# Autodesk Inventor assembly: launcher.motor
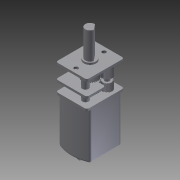
[picture p0: Inventor's stored thumbnail of the model, 180x180]
Saved by Autodesk Inventor 2011 (Build 150239000, 239)
## iProperties
Created: 2011-04-05
Part Number: launcher.motor
Document SubType Name: Assembly
Designer: Rob
Author: Rob
## Documents named in this file (5)
- C:\Users\M. Woods III\Desktop\design\Mechanical Drawings\launcher_motor.iam
- C:\Users\M. Woods III\Desktop\design\Mechanical Drawings\launcher_motor_main.ipt
- C:\Users\M. Woods III\Desktop\design\Mechanical Drawings\launcher_motor_shaft.ipt
- C:\Users\M. Woods III\Desktop\design\Mechanical Drawings\launcher_motor_midgear.ipt
- C:\Users\M. Woods III\Desktop\design\Mechanical Drawings\launcher_motor_lowgear.ipt
## Components (4 placed, 4 different names)
1. launcher_motor_main:1 — Mate:1, Mate:2, Mate:3, Mate:4, Mate:5, Mate:6, Mate:7
2. launcher_motor_shaft:1 — Mate:1, Mate:2, Mate:7, Rotation:1
3. launcher_motor_midgear:1 — Mate:3, Mate:4, Rotation:1, Rotation:2
4. launcher_motor_lowgear:1 — Mate:5, Mate:6, Rotation:2
## Relationships (9: Mate 7, RelateRotation 2)
- Mate:1: launcher_motor_main:1 ↔ launcher_motor_shaft:1
- Mate:2: launcher_motor_main:1 ↔ launcher_motor_shaft:1
- Mate:3: launcher_motor_main:1 ↔ launcher_motor_midgear:1
- Mate:4: launcher_motor_main:1 ↔ launcher_motor_midgear:1
- Mate:5: launcher_motor_main:1 ↔ launcher_motor_lowgear:1
- Mate:6: launcher_motor_main:1 ↔ launcher_motor_lowgear:1
- Mate:7: launcher_motor_main:1 ↔ launcher_motor_shaft:1
- Rotation:1 [RelateRotation] (2 ul): launcher_motor_shaft:1 ↔ launcher_motor_midgear:1
- Rotation:2 [RelateRotation] (0.3 ul): launcher_motor_midgear:1 ↔ launcher_motor_lowgear:1
